# Autodesk Inventor assembly: rotating_table
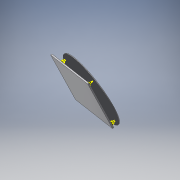
[picture p0: Inventor's stored thumbnail of the model, 180x180]
Saved by Autodesk Inventor 2016 (Build 200138000, 138)
## iProperties
Created: 2016-05-10
Part Number: rotating_table
Document SubType Name: Assembly
Designer: MAS Staff
Author: MAS Staff
## Documents named in this file (8)
- C:\Users\MAS Staff\Desktop\robocup-at-work\models\arena\elements\devices\rotating_turntable\inventor\rotating_table.iam
- C:\Users\MAS Staff\Desktop\robocup-at-work\models\arena\elements\devices\rotating_turntable\inventor\rotating_table_bottom_plate.ipt
- C:\Users\MAS Staff\Desktop\robocup-at-work\models\arena\elements\devices\rotating_turntable\inventor\rotating_table_shaft_plate.ipt
- C:\Users\MAS Staff\Desktop\robocup-at-work\models\arena\elements\devices\rotating_turntable\inventor\rotating_table_shaft.ipt
- C:\Users\MAS Staff\Desktop\robocup-at-work\models\arena\elements\devices\rotating_turntable\inventor\rotating_table_ball_bearing_holder.ipt
- C:\Users\MAS Staff\Desktop\robocup-at-work\models\arena\elements\devices\rotating_turntable\inventor\rotating_table_motor_holder.ipt
- C:\Users\MAS Staff\Desktop\robocup-at-work\models\arena\elements\devices\rotating_turntable\inventor\rotating_table_top_plate.ipt
- C:\Users\MAS Staff\Desktop\robocup-at-work\models\arena\elements\devices\rotating_turntable\inventor\rotating_table_belt_pulley_big.ipt
## Components (10 placed, 7 different names)
1. rotating_table_bottom_plate:1 — Mate:1, Mate:2, Mate:3, Mate:6, Mate:10, Mate:11, Mate:12, Mate:14, Mate:15, Mate:17, Mate:21, Mate:22, Mate:26, Mate:27, Mate:28, Mate:29
2. rotating_table_shaft_plate:1 — Mate:1, Mate:2, Mate:3, Mate:4, Mate:5, Mate:31, Mate:32
3. rotating_table_shaft:1 — Mate:4, Mate:5, Mate:35, Mate:36
4. rotating_table_ball_bearing_holder:1 — Mate:6, Mate:21, Mate:28
5. rotating_table_ball_bearing_holder:2 — Mate:11, Mate:14, Mate:27
6. rotating_table_ball_bearing_holder:3 — Mate:12, Mate:17, Mate:22
7. rotating_table_ball_bearing_holder:4 — Mate:10, Mate:15, Mate:26
8. rotating_table_motor_holder:1 — Mate:29, Mate:31, Mate:32
9. rotating_table_top_plate:1 — Mate:33, Mate:34, Mate:35, Mate:36
10. rotating_table_belt_pulley_big:1 — Mate:33, Mate:34
## Relationships (24: Mate 24)
- Mate:1: rotating_table_bottom_plate:1 ↔ rotating_table_shaft_plate:1
- Mate:2 (353.55 mm): rotating_table_bottom_plate:1 ↔ rotating_table_shaft_plate:1
- Mate:3 (-353.55 mm): rotating_table_bottom_plate:1 ↔ rotating_table_shaft_plate:1
- Mate:4: rotating_table_shaft_plate:1 ↔ rotating_table_shaft:1
- Mate:5: rotating_table_shaft_plate:1 ↔ rotating_table_shaft:1
- Mate:6: rotating_table_bottom_plate:1 ↔ rotating_table_ball_bearing_holder:1
- Mate:10: rotating_table_bottom_plate:1 ↔ rotating_table_ball_bearing_holder:4
- Mate:11: rotating_table_bottom_plate:1 ↔ rotating_table_ball_bearing_holder:2
- Mate:12: rotating_table_bottom_plate:1 ↔ rotating_table_ball_bearing_holder:3
- Mate:14 (20 mm): rotating_table_bottom_plate:1 ↔ rotating_table_ball_bearing_holder:2
- Mate:15 (20 mm): rotating_table_bottom_plate:1 ↔ rotating_table_ball_bearing_holder:4
- Mate:17 (20 mm): rotating_table_bottom_plate:1 ↔ rotating_table_ball_bearing_holder:3
- Mate:21 (20 mm): rotating_table_bottom_plate:1 ↔ rotating_table_ball_bearing_holder:1
- Mate:22 (687.1 mm): rotating_table_bottom_plate:1 ↔ rotating_table_ball_bearing_holder:3
- Mate:26 (687.1 mm): rotating_table_bottom_plate:1 ↔ rotating_table_ball_bearing_holder:4
- Mate:27 (20 mm): rotating_table_bottom_plate:1 ↔ rotating_table_ball_bearing_holder:2
- Mate:28 (20 mm): rotating_table_bottom_plate:1 ↔ rotating_table_ball_bearing_holder:1
- Mate:29: rotating_table_bottom_plate:1 ↔ rotating_table_motor_holder:1
- Mate:31: rotating_table_shaft_plate:1 ↔ rotating_table_motor_holder:1
- Mate:32 (-200 mm): rotating_table_shaft_plate:1 ↔ rotating_table_motor_holder:1
- Mate:33: rotating_table_top_plate:1 ↔ rotating_table_belt_pulley_big:1
- Mate:34: rotating_table_top_plate:1 ↔ rotating_table_belt_pulley_big:1
- Mate:35: rotating_table_shaft:1 ↔ rotating_table_top_plate:1
- Mate:36 (18 mm): rotating_table_shaft:1 ↔ rotating_table_top_plate:1
